# Autodesk Inventor assembly: Assembly2
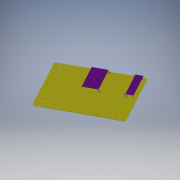
[picture p0: Inventor's stored thumbnail of the model, 180x180]
Saved by Autodesk Inventor 2019 (Build 230136000, 136)
## iProperties
Created: 2020-11-05
Part Number: Assembly2
Document SubType Name: Assembly
Designer: james
Author: james
## Documents named in this file (7)
- F:\JimsDesign\P1001-16bit-CPU\P1001-001 - 16bit CPU\P1001-001-004-320 - Register\Assembly2.iam
- F:\JimsDesign\P1001-16bit-CPU\P1001-001 - 16bit CPU\PRT1001-214 Base.ipt
- F:\JimsDesign\P1001-16bit-CPU\P1001-001 - 16bit CPU\P1001-001-004-320 - Register\Register.ipt
- F:\JimsDesign\P1001-16bit-CPU\P1001-001 - 16bit CPU\P1001-001-004-320 - Register\ALU.ipt
- F:\JimsDesign\P1001-16bit-CPU\P1001-001 - 16bit CPU\P1001-001-004-320 - Register\RAM.ipt
- F:\JimsDesign\P1001-16bit-CPU\P1001-001 - 16bit CPU\PRT1001-210 1U Board.ipt
- F:\JimsDesign\P1001-16bit-CPU\P1001-001 - 16bit CPU\PRT1001-211 2U Board.ipt
## Components (6 placed, 6 different names)
1. PRT1001-214 Base:1 — Mate:1, Mate:2, Mate:3, Mate:4, Mate:5, Mate:6, Mate:7, Mate:8, Mate:9
2. Register:1 — Mate:1, Mate:2, Mate:3, Mate:10, Mate:11, Mate:12
3. ALU:1 — Mate:4, Mate:5, Mate:6
4. RAM:1 — Mate:7, Mate:8, Mate:9, Mate:13, Mate:14, Mate:15
5. PRT1001-210 1U Board:1 — Mate:10, Mate:11, Mate:12
6. PRT1001-211 2U Board:1 — Mate:13, Mate:14, Mate:15
## Relationships (15: Mate 15)
- Mate:1: PRT1001-214 Base:1 ↔ Register:1
- Mate:2: PRT1001-214 Base:1 ↔ Register:1
- Mate:3: PRT1001-214 Base:1 ↔ Register:1
- Mate:4: PRT1001-214 Base:1 ↔ ALU:1
- Mate:5: PRT1001-214 Base:1 ↔ ALU:1
- Mate:6: PRT1001-214 Base:1 ↔ ALU:1
- Mate:7: PRT1001-214 Base:1 ↔ RAM:1
- Mate:8: PRT1001-214 Base:1 ↔ RAM:1
- Mate:9: PRT1001-214 Base:1 ↔ RAM:1
- Mate:10: Register:1 ↔ PRT1001-210 1U Board:1
- Mate:11: Register:1 ↔ PRT1001-210 1U Board:1
- Mate:12: Register:1 ↔ PRT1001-210 1U Board:1
- Mate:13: RAM:1 ↔ PRT1001-211 2U Board:1
- Mate:14: RAM:1 ↔ PRT1001-211 2U Board:1
- Mate:15: RAM:1 ↔ PRT1001-211 2U Board:1
